# Autodesk Inventor assembly: gear_mirrored
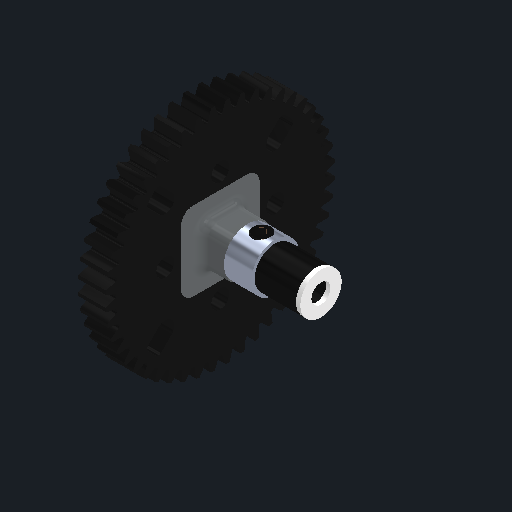
[picture p0: Inventor's stored thumbnail of the model, 512x512]
Saved by Autodesk Inventor 2025 (Build 290162000, 162)
## iProperties
Created: 2024-10-11
Part Number: gear_mirrored
Document SubType Name: Assembly
Designer: Averey Ku
Author: Averey Ku
## Documents named in this file (9)
- D:\vex_robotics_high_stakes\hardware\cad\bots\high_stakes_v2\chassis_v2\drivebay_mirrored\gear_mirrored.iam
- D:\vex_robotics_high_stakes\hardware\cad\bots\high_stakes_v2\chassis_v2\drivebay_mirrored\Half Cut HS 48T Gear, No Insert_mirrored.ipt
- D:\vex_robotics_high_stakes\hardware\cad\robpros_cad_lib\Motion\Spacers\Spacer Nylon .375 OD\NSpacer .375 OD x .375.ipt
- D:\vex_robotics_high_stakes\hardware\cad\robpros_cad_lib\Motion\Spacers\Spacer Nylon .375 OD.ipt
- D:\vex_robotics_high_stakes\hardware\cad\bots\high_stakes_v2\chassis_v2\drivebay_mirrored\Shaft Collar Set Screw_mirrored.ipt
- D:\vex_robotics_high_stakes\hardware\cad\robpros_cad_lib\Motion\Spacers\Washer Teflon\TWasher .375 OD x .04000.ipt
- D:\vex_robotics_high_stakes\hardware\cad\robpros_cad_lib\Motion\Spacers\Washer Teflon.ipt
- D:\vex_robotics_high_stakes\hardware\cad\robpros_cad_lib\Motion\Spacers\Washer Steel\SWasher .375 OD x .015625.ipt
- D:\vex_robotics_high_stakes\hardware\cad\robpros_cad_lib\Motion\Spacers\Washer Steel.ipt
## Components (5 placed, 5 different names)
1. Half Cut HS 48T Gear, No Insert_mirrored:1 — Mate:1, Insert:4, Insert:1
2. NSpacer .375 OD x .375:1 — Insert:2, Insert:3
3. Shaft Collar Set Screw_mirrored:1 — Insert:4, Insert:2
4. TWasher .375 OD x .04000:1 — Insert:3
5. SWasher .375 OD x .015625:1 — Insert:1
## Relationships (5: Insert 4, Mate 1)
- Mate:1: Half Cut HS 48T Gear, No Insert_mirrored:1
- Insert:4: Half Cut HS 48T Gear, No Insert_mirrored:1 ↔ Shaft Collar Set Screw_mirrored:1
- Insert:2: NSpacer .375 OD x .375:1 ↔ Shaft Collar Set Screw_mirrored:1
- Insert:3: NSpacer .375 OD x .375:1 ↔ TWasher .375 OD x .04000:1
- Insert:1: Half Cut HS 48T Gear, No Insert_mirrored:1 ↔ SWasher .375 OD x .015625:1
